# Autodesk Inventor assembly: StraightPumpRegion
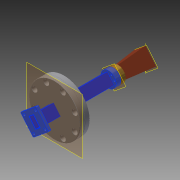
[picture p0: Inventor's stored thumbnail of the model, 180x180]
Saved by Autodesk Inventor 2015 (Build 190159000, 159)
## iProperties
Created: 2014-03-24
Part Number: StraightPumpRegion
Document SubType Name: Assembly
Designer: jad211
Author: jad211
## Documents named in this file (5)
- C:\CADFiles\EDM Machine\EDM New Pumping Region\StraightPumpRegion.iam
- C:\CADFiles\EDM Machine\EDM New Pumping Region\NewHorn.ipt
- C:\CADFiles\EDM Machine\EDM New Pumping Region\WG18FLANGECutDown.ipt
- C:\CADFiles\EDM Machine\EDM New Pumping Region\FlangedWaveguide.iam
- C:\CADFiles\EDM Machine\EDM New Pumping Region\3-38sWithWG18Hole.ipt
## Components (4 placed, 4 different names)
1. NewHorn:1 — Angle:2, Flush:17, Mate:17, Mate:18, Mate:19, Mate:21, Flush:20
2. WG18FLANGECutDown:1 — Flush:17, Mate:18, Mate:19, Mate:20
3. FlangedWaveguide:2 [sub-assembly] — Mate:17, Mate:20, Mate:21, Mate:22, Mate:23
4. 3-38sWithWG18Hole:1 — Mate:22, Mate:23
## Relationships (10: Mate 7, Flush 2, Angle 1)
- Angle:2 (0 deg): NewHorn:1
- Flush:17: NewHorn:1 ↔ WG18FLANGECutDown:1
- Mate:17: NewHorn:1 ↔ FlangedWaveguide:2
- Mate:18: NewHorn:1 ↔ WG18FLANGECutDown:1
- Mate:19: NewHorn:1 ↔ WG18FLANGECutDown:1
- Mate:20: WG18FLANGECutDown:1 ↔ FlangedWaveguide:2
- Mate:21: NewHorn:1 ↔ FlangedWaveguide:2
- Flush:20 (-5 mm): NewHorn:1
- Mate:22: FlangedWaveguide:2 ↔ 3-38sWithWG18Hole:1
- Mate:23: FlangedWaveguide:2 ↔ 3-38sWithWG18Hole:1
